# Autodesk Inventor assembly: Assembly ebeam heater IS v0
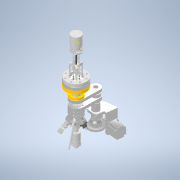
[picture p0: Inventor's stored thumbnail of the model, 180x180]
Saved by Autodesk Inventor 2020 (Build 240168000, 168)
## iProperties
Created: 2019-05-26
Part Number: Assembly ebeam heater IS v0
Document SubType Name: Assembly
Designer: isadmin
Mass: 1360.95 g
Surface Area: 5412.04 cm^2
Volume: 1345.69 cm^3
Density: 1.01134 g/cm^3
Author: isadmin
## Documents named in this file (42)
- C:\Users\ColinP\Documents\Inventor\igor\Assembly ebeam heater CP v3.iam
- Assembly ebeam heater IS v0.iam
- C:\Users\ColinP\Documents\Inventor\igor\block.ipt
- C:\Users\ColinP\Documents\Inventor\igor\Shutter.ipt
- C:\Users\ColinP\Documents\Inventor\igor\ceramic washer.ipt
- C:\Users\ColinP\Documents\Inventor\igor\Shielding.ipt
- C:\Users\ColinP\Documents\Inventor\igor\Bullet_v5_SiliconeSample.ipt
- C:\Users\ColinP\Documents\Inventor\igor\Bullet_v5_SiliconeSample_TopPart.ipt
- C:\Users\ColinP\Documents\Inventor\igor\670000.ipt
- C:\Users\ColinP\Documents\Inventor\igor\MCF275-FlgMplxr-Cr1A5_(53-321020-A).ipt
- C:\Users\ColinP\Documents\Inventor\igor\665501.ipt
- C:\Users\ColinP\Documents\Inventor\igor\rotatable rod table.ipt
- C:\Users\ColinP\Documents\Inventor\igor\updated table+legs.iam
- C:\Users\ColinP\Documents\Inventor\igor\square eyelet.ipt
- C:\Users\ColinP\Documents\Inventor\igor\buffer.ipt
- C:\Users\ColinP\Documents\Inventor\igor\4.5to2.75converotr.ipt
- C:\Users\ColinP\Documents\Inventor\igor\rotaryconnector.ipt
- C:\Users\ColinP\Documents\Inventor\igor\140007.ipt
- C:\Users\ColinP\Documents\Inventor\Content Center Files\R2020\en-US\ISO 4029\ISO 4029 - M2 x 2 - ISO.ipt
- C:\Users\ColinP\Documents\Inventor\igor\9312007.iam
- C:\Users\ColinP\Documents\Inventor\igor\eft0181032.ipt
- C:\Users\ColinP\Documents\Inventor\igor\filwasher.ipt
- C:\Users\ColinP\Documents\Inventor\igor\fileholddub.ipt
- C:\Users\ColinP\Documents\Inventor\Content Center Files\R2020\en-US\ISO 4017(1)\ISO 4017 - M2.5 x 5 - ISO.ipt
- C:\Users\ColinP\Documents\Inventor\igor\water.ipt
- C:\Users\ColinP\Documents\Inventor\igor\stability copy2.ipt
- C:\Users\ColinP\Documents\Inventor\igor\stability copy.ipt
- C:\Users\ColinP\Documents\Inventor\igor\shroud 2.ipt
- C:\Users\ColinP\Documents\Inventor\igor\4.5 rod.ipt
- C:\Users\ColinP\Documents\Inventor\igor\5011T170_WORM-DRIVE CLAMP FOR FIRM HOSE AND TUBE.ipt
- C:\Users\ColinP\Documents\Inventor\igor\filament.ipt
- C:\Users\ColinP\Documents\Inventor\Content Center Files\R2020\en-US\ISO 4032(2)\ISO 4032 - M3.5 - ISO.ipt
- C:\Users\ColinP\Documents\Inventor\igor\110001.ipt
- C:\Users\ColinP\Documents\Inventor\igor\waterpipe assembly.ipt
- C:\Users\ColinP\Documents\Inventor\igor\waterpipe assembly 2.ipt
- C:\Users\ColinP\Documents\Inventor\igor\waterpipe3.ipt
- C:\Users\ColinP\Documents\Inventor\igor\flange 4_5 double_sided.ipt
- C:\Users\ColinP\Downloads\SS-2-VCR-CG-SwagelokCompany-07-31-2019(1).ipt
- C:\Users\ColinP\Downloads\SS-2-VCR-1-2-SwagelokCompany-08-01-2019.ipt
- C:\Users\ColinP\Documents\Inventor\Content Center Files\R2020\en-US\ISO 4032(2)\ISO 4032 - M3 - ISO.ipt
- C:\Users\ColinP\Downloads\110021.ipt
- C:\Users\ColinP\Documents\Inventor\igor\part12.ipt
## Components (150 placed, 40 different names)
1. rotatable rod table:1 — Mate:48, Insert:171, Insert:173, Insert:174, Insert:175, Rigid:18, Insert:176, Insert:177, Insert:181, Insert:187, Mate:246, Insert:207, Mate:273, Mate:274
2. block for bullet:1 — Mate:249
3. Shutter:1
4. ceramic washer:1
5. ceramic washer:2
6. ceramic washer:3
7. ceramic washer:4
8. Shielding:1
9. ceramic washer:5
10. ceramic washer:6
11. ceramic washer:7
12. ceramic washer:8
13. Bullet_v5_SiliconeSample:1
14. Bullet_v5_SiliconeSample_TopPart:1
15. rotation_670000:1 — Rotational:3, Rigid:18
16. MCF275-FlgMplxr-Cr1A5_(53-321020-A):1 — Rotational:3, Rigid:5, Rotational:14, Rotational:16, Rigid:23, Rigid:24
17. zstage_665501:1 — Rigid:8, Cylindrical:1, Mate:235
18. 140007:1 — Rigid:5, Rigid:8, Insert:131, Insert:132, Insert:133, Insert:134, Insert:135, Insert:136, Mate:272, Mate:396, Mate:398
19. updated table+legs:1 [sub-assembly] — Mate:48, Mate:72, Rigid:14, Insert:166, Angle:1, Mate:215, Mate:216, Mate:217, Mate:218, Mate:219, Mate:220, Rotational:12, Rigid:22, Mate:241, Mate:250, Mate:254, Mate:278, Mate:281, Mate:288, Mate:290, Mate:292, Mate:294, Mate:296, Mate:298, Mate:300, Mate:302, Mate:304, Mate:306, Mate:308, Mate:310, Mate:312, Mate:314, Mate:316, Mate:318, Mate:320, Mate:322, Mate:324, Mate:326, Mate:328, Mate:330, Mate:332, Mate:334, Mate:336, Mate:338, Mate:340, Mate:342, Mate:344, Mate:346, Mate:348, Mate:350, Mate:352, Mate:354, Mate:356, Mate:358, Mate:360, Mate:362, Mate:364, Mate:366, Mate:368, Mate:370, Mate:404, Mate:406, Mate:408, Mate:430, Mate:432, Mate:434, Mate:436
20. buffer:4 — Insert:173
21. square eyelet:24 — Mate:327, Mate:339
22. square eyelet:25 — Mate:218, Mate:329, Mate:331
23. square eyelet:26 — Mate:325, Mate:337
24. buffer:5 — Insert:171
25. square eyelet:27 — Mate:349, Mate:363
26. square eyelet:28 — Mate:216, Mate:351, Mate:355
27. square eyelet:29 — Mate:353, Mate:357
28. buffer:6 — Insert:161, Insert:162, Insert:163, Insert:174
29. buffer:7 — Insert:176
30. square eyelet:33 — Mate:293, Mate:295
31. square eyelet:34 — Mate:220, Mate:297, Mate:299
32. square eyelet:35 — Mate:289, Mate:291
33. buffer:9 — Insert:177
34. square eyelet:39 — Mate:341, Mate:347
35. square eyelet:40 — Mate:217, Mate:333, Mate:343
36. square eyelet:41 — Mate:335, Mate:345
37. rotaryconnector:2 — Insert:149, Insert:150, Insert:151, Insert:152, Insert:187
38. square eyelet:49 — Insert:134, Mate:437
39. square eyelet:50 — Insert:135, Mate:435
40. square eyelet:51 — Insert:133, Insert:222
41. square eyelet:52 — Insert:131, Mate:72, Mate:433
42. square eyelet:53 — Insert:132, Mate:431
43. square eyelet:54 — Insert:136, Insert:223
44. buffer:10 — Insert:175
45. square eyelet:55 — Mate:215, Mate:315, Mate:323
46. square eyelet:56 — Mate:313, Mate:321
47. square eyelet:57 — Mate:317, Mate:319
48. 9312007:1 [sub-assembly] — Rotational:16
49. eft0181032:1 — Rigid:23
50. square eyelet:64 — Insert:162, Mate:301, Mate:303
51. square eyelet:65 — Insert:163, Mate:305, Mate:307
52. square eyelet:66 — Insert:161, Mate:219, Mate:309, Mate:311
53. filwasher:2 — Rigid:14, Insert:168, Rotational:12, Mate:279
54. fileholddub:1 — Insert:166, Rigid:17, Rotational:9, Angle:1
55. filwasher:5 — Rotational:9, Insert:169, Mate:280
56. filwasher:6 — Rigid:17, Insert:170, Mate:277
57. filwasher:7 — Insert:167, Rigid:22, Mate:276
58. buffer:11 — Insert:178, Insert:179, Insert:180, Insert:181
59. square eyelet:67 — Insert:178, Mate:361, Mate:367
60. square eyelet:68 — Insert:179, Mate:359, Mate:371
61. square eyelet:69 — Insert:180, Mate:254, Mate:365, Mate:369
62. ISO 4029 M2 x 2:1 — Insert:152
63. ISO 4029 M2 x 2:2 — Insert:150
64. ISO 4029 M2 x 2:3 — Insert:151
65. ISO 4029 M2 x 2:4 — Insert:149
66. ISO 4017 M2.5 x 5:1 — Insert:167
67. ISO 4017 M2.5 x 5:2 — Insert:168
68. ISO 4017 M2.5 x 5:3 — Insert:169
69. ISO 4017 M2.5 x 5:4 — Insert:170
70. water:1 — Insert:207, Insert:208, Insert:209, Insert:210, Flush:267, Mate:405, Mate:407, Mate:409, Mate:440, Mate:443, Insert:224, Insert:225
71. square eyelet:70 — Insert:210
72. square eyelet:71 — Insert:208, Mate:250
73. square eyelet:72 — Insert:209
74. 4.5to2.75converotr:1 — Cylindrical:1, Mate:235, Rigid:25
75. shroud 2:1 — Mate:241, Mate:249, Mate:264
76. 4.5 rod:1 — Mate:247, Mate:248, Insert:219
77. 4.5 rod:2 — Insert:221
78. 4.5 rod:3 — Insert:220
79. stability copy:1 — Insert:204, Insert:205, Insert:206, Mate:243, Mate:244, Mate:245, Mate:246
80. stability copy2:1 — Insert:205, Mate:244, Mate:247, Mate:248, Mate:286
81. stability copy2:2 — Insert:206, Mate:245, Mate:287
82. stability copy2:3 — Insert:204, Mate:243
83. 5011T170_WORM-DRIVE CLAMP FOR FIRM HOSE AND TUBE:1 — Mate:264, Flush:267
84. filament:1 — Mate:279, Mate:280, Mate:281
85. filament:2 — Mate:276, Mate:277, Mate:278
86. ISO 4032 M3.5:1 — Mate:288, Mate:289
87. ISO 4032 M3.5:2 — Mate:290, Mate:291
88. ISO 4032 M3.5:3 — Mate:292, Mate:293
89. ISO 4032 M3.5:4 — Mate:294, Mate:295
90. ISO 4032 M3.5:5 — Mate:296, Mate:297
91. ISO 4032 M3.5:6 — Mate:298, Mate:299
92. ISO 4032 M3.5:7 — Mate:300, Mate:301
93. ISO 4032 M3.5:8 — Mate:302, Mate:303
94. ISO 4032 M3.5:9 — Mate:304, Mate:305
95. ISO 4032 M3.5:10 — Mate:306, Mate:307
96. ISO 4032 M3.5:11 — Mate:308, Mate:309
97. ISO 4032 M3.5:12 — Mate:310, Mate:311
98. ISO 4032 M3.5:13 — Mate:312, Mate:313
99. ISO 4032 M3.5:14 — Mate:314, Mate:315
100. ISO 4032 M3.5:15 — Mate:316, Mate:317
101. ISO 4032 M3.5:16 — Mate:318, Mate:319
102. ISO 4032 M3.5:17 — Mate:320, Mate:321
103. ISO 4032 M3.5:18 — Mate:322, Mate:323
104. ISO 4032 M3.5:19 — Mate:324, Mate:325
105. ISO 4032 M3.5:20 — Mate:326, Mate:327
106. ISO 4032 M3.5:21 — Mate:328, Mate:329
107. ISO 4032 M3.5:22 — Mate:330, Mate:331
108. ISO 4032 M3.5:23 — Mate:332, Mate:333
109. ISO 4032 M3.5:24 — Mate:334, Mate:335
110. ISO 4032 M3.5:25 — Mate:336, Mate:337
111. ISO 4032 M3.5:26 — Mate:338, Mate:339
112. ISO 4032 M3.5:27 — Mate:340, Mate:341
113. ISO 4032 M3.5:28 — Mate:342, Mate:343
114. ISO 4032 M3.5:29 — Mate:344, Mate:345
115. ISO 4032 M3.5:30 — Mate:346, Mate:347
116. ISO 4032 M3.5:31 — Mate:348, Mate:349
117. ISO 4032 M3.5:32 — Mate:350, Mate:351
118. ISO 4032 M3.5:33 — Mate:352, Mate:353
119. ISO 4032 M3.5:34 — Mate:354, Mate:355
120. ISO 4032 M3.5:35 — Mate:356, Mate:357
121. ISO 4032 M3.5:36 — Mate:358, Mate:359
122. ISO 4032 M3.5:37 — Mate:360, Mate:361
123. ISO 4032 M3.5:38 — Mate:362, Mate:363
124. ISO 4032 M3.5:39 — Mate:364, Mate:365
125. ISO 4032 M3.5:40 — Mate:366, Mate:367
126. ISO 4032 M3.5:41 — Mate:368, Mate:369
127. ISO 4032 M3.5:42 — Mate:370, Mate:371
128. 110001:1 — Rotational:14, Mate:397
129. 110001:2 — Rigid:24, Mate:399
130. waterpipe assembly:1 — Mate:396, Mate:397, Mate:410, Mate:411, Mate:429
131. waterpipe assembly 2:1 — Mate:398, Mate:399, Mate:412, Mate:413, Mate:428
132. ISO 4032 M3.5:55 — Mate:404, Mate:405
133. ISO 4032 M3.5:56 — Mate:406, Mate:407
134. ISO 4032 M3.5:57 — Mate:408, Mate:409
135. waterpipe3:1 — Mate:410, Mate:411, Mate:429, Mate:439
136. waterpipe3:2 — Mate:412, Mate:413, Mate:428, Mate:438
137. flange 4_5 double_sided:1 — Rigid:25, Insert:219, Insert:220, Insert:221, Rigid:26
138. SS-2-VCR-CG-SwagelokCompany-07-31-2019(1):1 — Mate:418, Mate:419, Mate:439
139. SS-2-VCR-CG-SwagelokCompany-07-31-2019(1):2 — Mate:420, Mate:421, Mate:438
140. SS-2-VCR-1-2-SwagelokCompany-08-01-2019:1 — Mate:418, Mate:419, Mate:444
141. SS-2-VCR-1-2-SwagelokCompany-08-01-2019:2 — Mate:420, Mate:421, Mate:445
142. ISO 4032 M3.5:58 — Mate:430, Mate:431
143. ISO 4032 M3:1 — Insert:222
144. ISO 4032 M3.5:59 — Mate:432, Mate:433
145. ISO 4032 M3:2 — Insert:223
146. ISO 4032 M3:3 — Mate:434, Mate:435
147. ISO 4032 M3:4 — Mate:436, Mate:437
148. 110021:1 — Rigid:26
149. part12:1 — Mate:443, Insert:224, Mate:444, Symmetry:1
150. part12:2 — Mate:440, Insert:225, Mate:445, Symmetry:1
## Relationships (254: Mate 171, Insert 61, WeldJoint 10, RevoluteJoint 5, Flush 4, Angle 1, CylindricalJoint 1, Symmetry 1)
- [Mate]: block for bullet:1 ↔ Shutter:1
- [Mate]: block for bullet:1 ↔ Shutter:1
- [Mate]: block for bullet:1 ↔ Shutter:1
- [Mate]: block for bullet:1 ↔ ceramic washer:2
- [Mate]: block for bullet:1 ↔ ceramic washer:2
- [Mate]: block for bullet:1 ↔ ceramic washer:1
- [Mate]: block for bullet:1 ↔ ceramic washer:1
- [Mate]: block for bullet:1 ↔ ceramic washer:4
- [Mate]: block for bullet:1 ↔ ceramic washer:4
- [Mate]: block for bullet:1 ↔ ceramic washer:3
- [Mate]: block for bullet:1 ↔ ceramic washer:3
- [Mate]: ceramic washer:1 ↔ Shielding:1
- [Flush]: block for bullet:1 ↔ Shielding:1
- [Flush]: block for bullet:1 ↔ Shielding:1
- [Mate]: block for bullet:1 ↔ ceramic washer:5
- [Mate]: block for bullet:1 ↔ ceramic washer:5
- [Mate]: block for bullet:1 ↔ ceramic washer:6
- [Mate]: block for bullet:1 ↔ ceramic washer:6
- [Mate]: block for bullet:1 ↔ ceramic washer:7
- [Mate]: block for bullet:1 ↔ ceramic washer:7
- [Mate]: block for bullet:1 ↔ ceramic washer:8
- [Mate]: block for bullet:1 ↔ ceramic washer:8
- [Mate] (0.0254 mm): Bullet_v5_SiliconeSample:1 ↔ Bullet_v5_SiliconeSample_TopPart:1
- [Mate]: Bullet_v5_SiliconeSample:1 ↔ Bullet_v5_SiliconeSample_TopPart:1
- [Insert]: block for bullet:1 ↔ Bullet_v5_SiliconeSample:1
- [Insert]: rotatable rod table:1 ↔ block for bullet:1
- [Insert]: rotatable rod table:1 ↔ block for bullet:1
- [Insert]: buffer:4 ↔ square eyelet:25
- [Insert]: buffer:4 ↔ square eyelet:24
- [Insert]: buffer:4 ↔ square eyelet:26
- [Insert]: buffer:5 ↔ square eyelet:28
- [Insert]: buffer:5 ↔ square eyelet:27
- [Insert]: buffer:5 ↔ square eyelet:29
- [Insert]: buffer:7 ↔ square eyelet:34
- [Insert]: buffer:7 ↔ square eyelet:33
- [Insert]: buffer:7 ↔ square eyelet:35
- [Insert]: buffer:9 ↔ square eyelet:40
- [Insert]: buffer:9 ↔ square eyelet:39
- [Insert]: buffer:9 ↔ square eyelet:41
- Mate:48: rotatable rod table:1 ↔ updated table+legs:1
- Rotational:3 [RevoluteJoint]: rotation_670000:1 ↔ MCF275-FlgMplxr-Cr1A5_(53-321020-A):1
- Rigid:5 [WeldJoint]: MCF275-FlgMplxr-Cr1A5_(53-321020-A):1 ↔ 140007:1
- Rigid:8 [WeldJoint]: zstage_665501:1 ↔ 140007:1
- Insert:131: 140007:1 ↔ square eyelet:52
- Insert:132: 140007:1 ↔ square eyelet:53
- Insert:133: 140007:1 ↔ square eyelet:51
- Insert:134: 140007:1 ↔ square eyelet:49
- Insert:135: 140007:1 ↔ square eyelet:50
- Insert:136: 140007:1 ↔ square eyelet:54
- [Insert]: buffer:10 ↔ square eyelet:56
- [Insert]: buffer:10 ↔ square eyelet:55
- [Insert]: buffer:10 ↔ square eyelet:57
- Insert:149: rotaryconnector:2 ↔ ISO 4029 M2 x 2:4
- Insert:150: rotaryconnector:2 ↔ ISO 4029 M2 x 2:2
- Insert:151: rotaryconnector:2 ↔ ISO 4029 M2 x 2:3
- Insert:152: rotaryconnector:2 ↔ ISO 4029 M2 x 2:1
- Mate:72: updated table+legs:1 ↔ square eyelet:52
- Insert:161: buffer:6 ↔ square eyelet:66
- Insert:162: buffer:6 ↔ square eyelet:64
- Insert:163: buffer:6 ↔ square eyelet:65
- Rigid:14 [WeldJoint]: updated table+legs:1 ↔ filwasher:2
- Insert:166 (-6.35 mm): updated table+legs:1 ↔ fileholddub:1
- Rigid:17 [WeldJoint]: fileholddub:1 ↔ filwasher:6
- Rotational:9 [RevoluteJoint]: fileholddub:1 ↔ filwasher:5
- Insert:167: filwasher:7 ↔ ISO 4017 M2.5 x 5:1
- Insert:168: filwasher:2 ↔ ISO 4017 M2.5 x 5:2
- Insert:169: filwasher:5 ↔ ISO 4017 M2.5 x 5:3
- Insert:170: filwasher:6 ↔ ISO 4017 M2.5 x 5:4
- Insert:171 (175.895 mm): rotatable rod table:1 ↔ buffer:5
- Insert:173 (199.644 mm): rotatable rod table:1 ↔ buffer:4
- Insert:174 (223.52 mm): rotatable rod table:1 ↔ buffer:6
- Insert:175 (211.455 mm): rotatable rod table:1 ↔ buffer:10
- Angle:1 (180 deg): updated table+legs:1 ↔ fileholddub:1
- Rigid:18 [WeldJoint]: rotatable rod table:1 ↔ rotation_670000:1
- Insert:176 (235.585 mm): rotatable rod table:1 ↔ buffer:7
- Insert:177 (187.96 mm): rotatable rod table:1 ↔ buffer:9
- Insert:178: buffer:11 ↔ square eyelet:67
- Insert:179: buffer:11 ↔ square eyelet:68
- Insert:180: buffer:11 ↔ square eyelet:69
- Insert:181 (163.83 mm): rotatable rod table:1 ↔ buffer:11
- Insert:187 (-12.7 mm): rotatable rod table:1 ↔ rotaryconnector:2
- Cylindrical:1: zstage_665501:1 ↔ 4.5to2.75converotr:1
- Mate:215: updated table+legs:1 ↔ square eyelet:55
- Mate:216: updated table+legs:1 ↔ square eyelet:28
- Mate:217: updated table+legs:1 ↔ square eyelet:40
- Mate:218: updated table+legs:1 ↔ square eyelet:25
- Mate:219: updated table+legs:1 ↔ square eyelet:66
- Mate:220: updated table+legs:1 ↔ square eyelet:34
- Rotational:12 [RevoluteJoint]: updated table+legs:1 ↔ filwasher:2
- Rigid:22 [WeldJoint]: updated table+legs:1 ↔ filwasher:7
- Mate:235: zstage_665501:1 ↔ 4.5to2.75converotr:1
- Mate:241: updated table+legs:1 ↔ shroud 2:1
- Insert:204: stability copy:1 ↔ stability copy2:3
- Insert:205: stability copy:1 ↔ stability copy2:1
- Insert:206: stability copy:1 ↔ stability copy2:2
- Mate:243: stability copy:1 ↔ stability copy2:3
- Mate:244: stability copy:1 ↔ stability copy2:1
- Mate:245: stability copy:1 ↔ stability copy2:2
- Mate:246: rotatable rod table:1 ↔ stability copy:1
- Mate:247: 4.5 rod:1 ↔ stability copy2:1
- Mate:248: 4.5 rod:1 ↔ stability copy2:1
- Mate:249: block for bullet:1 ↔ shroud 2:1
- Insert:207 (27.94 mm): rotatable rod table:1 ↔ water:1
- Insert:208: water:1 ↔ square eyelet:71
- Insert:209: water:1 ↔ square eyelet:72
- Insert:210: water:1 ↔ square eyelet:70
- Mate:250: updated table+legs:1 ↔ square eyelet:71
- Mate:254: updated table+legs:1 ↔ square eyelet:69
- Mate:264: shroud 2:1 ↔ 5011T170_WORM-DRIVE CLAMP FOR FIRM HOSE AND TUBE:1
- Mate:272: 140007:1
- Mate:273: rotatable rod table:1
- Mate:274: rotatable rod table:1
- Mate:276: filwasher:7 ↔ filament:2
- Mate:277: filwasher:6 ↔ filament:2
- Mate:278: updated table+legs:1 ↔ filament:2
- Mate:279: filwasher:2 ↔ filament:1
- Mate:280: filwasher:5 ↔ filament:1
- Mate:281: updated table+legs:1 ↔ filament:1
- Mate:286: stability copy2:1
- Mate:287: stability copy2:2
- Mate:288: updated table+legs:1 ↔ ISO 4032 M3.5:1
- Mate:289: square eyelet:35 ↔ ISO 4032 M3.5:1
- Mate:290: updated table+legs:1 ↔ ISO 4032 M3.5:2
- Mate:291: square eyelet:35 ↔ ISO 4032 M3.5:2
- Mate:292: updated table+legs:1 ↔ ISO 4032 M3.5:3
- Mate:293: square eyelet:33 ↔ ISO 4032 M3.5:3
- Mate:294: updated table+legs:1 ↔ ISO 4032 M3.5:4
- Mate:295: square eyelet:33 ↔ ISO 4032 M3.5:4
- Mate:296: updated table+legs:1 ↔ ISO 4032 M3.5:5
- Mate:297: square eyelet:34 ↔ ISO 4032 M3.5:5
- Mate:298: updated table+legs:1 ↔ ISO 4032 M3.5:6
- Mate:299: square eyelet:34 ↔ ISO 4032 M3.5:6
- Mate:300: updated table+legs:1 ↔ ISO 4032 M3.5:7
- Mate:301: square eyelet:64 ↔ ISO 4032 M3.5:7
- Mate:302: updated table+legs:1 ↔ ISO 4032 M3.5:8
- Mate:303: square eyelet:64 ↔ ISO 4032 M3.5:8
- Mate:304: updated table+legs:1 ↔ ISO 4032 M3.5:9
- Mate:305: square eyelet:65 ↔ ISO 4032 M3.5:9
- Mate:306: updated table+legs:1 ↔ ISO 4032 M3.5:10
- Mate:307: square eyelet:65 ↔ ISO 4032 M3.5:10
- Mate:308: updated table+legs:1 ↔ ISO 4032 M3.5:11
- Mate:309: square eyelet:66 ↔ ISO 4032 M3.5:11
- Mate:310: updated table+legs:1 ↔ ISO 4032 M3.5:12
- Mate:311: square eyelet:66 ↔ ISO 4032 M3.5:12
- Mate:312: updated table+legs:1 ↔ ISO 4032 M3.5:13
- Mate:313: square eyelet:56 ↔ ISO 4032 M3.5:13
- Mate:314: updated table+legs:1 ↔ ISO 4032 M3.5:14
- Mate:315: square eyelet:55 ↔ ISO 4032 M3.5:14
- Mate:316: updated table+legs:1 ↔ ISO 4032 M3.5:15
- Mate:317: square eyelet:57 ↔ ISO 4032 M3.5:15
- Mate:318: updated table+legs:1 ↔ ISO 4032 M3.5:16
- Mate:319: square eyelet:57 ↔ ISO 4032 M3.5:16
- Mate:320: updated table+legs:1 ↔ ISO 4032 M3.5:17
- Mate:321: square eyelet:56 ↔ ISO 4032 M3.5:17
- Mate:322: updated table+legs:1 ↔ ISO 4032 M3.5:18
- Mate:323: square eyelet:55 ↔ ISO 4032 M3.5:18
- Mate:324: updated table+legs:1 ↔ ISO 4032 M3.5:19
- Mate:325: square eyelet:26 ↔ ISO 4032 M3.5:19
- Mate:326: updated table+legs:1 ↔ ISO 4032 M3.5:20
- Mate:327: square eyelet:24 ↔ ISO 4032 M3.5:20
- Mate:328: updated table+legs:1 ↔ ISO 4032 M3.5:21
- Mate:329: square eyelet:25 ↔ ISO 4032 M3.5:21
- Mate:330: updated table+legs:1 ↔ ISO 4032 M3.5:22
- Mate:331: square eyelet:25 ↔ ISO 4032 M3.5:22
- Mate:332: updated table+legs:1 ↔ ISO 4032 M3.5:23
- Mate:333: square eyelet:40 ↔ ISO 4032 M3.5:23
- Mate:334: updated table+legs:1 ↔ ISO 4032 M3.5:24
- Mate:335: square eyelet:41 ↔ ISO 4032 M3.5:24
- Mate:336: updated table+legs:1 ↔ ISO 4032 M3.5:25
- Mate:337: square eyelet:26 ↔ ISO 4032 M3.5:25
- Mate:338: updated table+legs:1 ↔ ISO 4032 M3.5:26
- Mate:339: square eyelet:24 ↔ ISO 4032 M3.5:26
- Mate:340: updated table+legs:1 ↔ ISO 4032 M3.5:27
- Mate:341: square eyelet:39 ↔ ISO 4032 M3.5:27
- Mate:342: updated table+legs:1 ↔ ISO 4032 M3.5:28
- Mate:343: square eyelet:40 ↔ ISO 4032 M3.5:28
- Mate:344: updated table+legs:1 ↔ ISO 4032 M3.5:29
- Mate:345: square eyelet:41 ↔ ISO 4032 M3.5:29
- Mate:346: updated table+legs:1 ↔ ISO 4032 M3.5:30
- Mate:347: square eyelet:39 ↔ ISO 4032 M3.5:30
- Mate:348: updated table+legs:1 ↔ ISO 4032 M3.5:31
- Mate:349: square eyelet:27 ↔ ISO 4032 M3.5:31
- Mate:350: updated table+legs:1 ↔ ISO 4032 M3.5:32
- Mate:351: square eyelet:28 ↔ ISO 4032 M3.5:32
- Mate:352: updated table+legs:1 ↔ ISO 4032 M3.5:33
- Mate:353: square eyelet:29 ↔ ISO 4032 M3.5:33
- Mate:354: updated table+legs:1 ↔ ISO 4032 M3.5:34
- Mate:355: square eyelet:28 ↔ ISO 4032 M3.5:34
- Mate:356: updated table+legs:1 ↔ ISO 4032 M3.5:35
- Mate:357: square eyelet:29 ↔ ISO 4032 M3.5:35
- Mate:358: updated table+legs:1 ↔ ISO 4032 M3.5:36
- Mate:359: square eyelet:68 ↔ ISO 4032 M3.5:36
- Mate:360: updated table+legs:1 ↔ ISO 4032 M3.5:37
- Mate:361: square eyelet:67 ↔ ISO 4032 M3.5:37
- Mate:362: updated table+legs:1 ↔ ISO 4032 M3.5:38
- Mate:363: square eyelet:27 ↔ ISO 4032 M3.5:38
- Mate:364: updated table+legs:1 ↔ ISO 4032 M3.5:39
- Mate:365: square eyelet:69 ↔ ISO 4032 M3.5:39
- Mate:366: updated table+legs:1 ↔ ISO 4032 M3.5:40
- Mate:367: square eyelet:67 ↔ ISO 4032 M3.5:40
- Mate:368: updated table+legs:1 ↔ ISO 4032 M3.5:41
- Mate:369: square eyelet:69 ↔ ISO 4032 M3.5:41
- Mate:370: updated table+legs:1 ↔ ISO 4032 M3.5:42
- Mate:371: square eyelet:68 ↔ ISO 4032 M3.5:42
- Rotational:14 [RevoluteJoint]: MCF275-FlgMplxr-Cr1A5_(53-321020-A):1 ↔ 110001:1
- Rotational:16 [RevoluteJoint]: MCF275-FlgMplxr-Cr1A5_(53-321020-A):1 ↔ 9312007:1
- Rigid:23 [WeldJoint]: MCF275-FlgMplxr-Cr1A5_(53-321020-A):1 ↔ eft0181032:1
- Rigid:24 [WeldJoint]: MCF275-FlgMplxr-Cr1A5_(53-321020-A):1 ↔ 110001:2
- Flush:3 (3.175 mm)
- Mate:396: 140007:1 ↔ waterpipe assembly:1
- Mate:397: 110001:1 ↔ waterpipe assembly:1
- Mate:398: 140007:1 ↔ waterpipe assembly 2:1
- Mate:399: 110001:2 ↔ waterpipe assembly 2:1
- Flush:267: water:1 ↔ 5011T170_WORM-DRIVE CLAMP FOR FIRM HOSE AND TUBE:1
- Mate:404: updated table+legs:1 ↔ ISO 4032 M3.5:55
- Mate:405: water:1 ↔ ISO 4032 M3.5:55
- Mate:406: updated table+legs:1 ↔ ISO 4032 M3.5:56
- Mate:407: water:1 ↔ ISO 4032 M3.5:56
- Mate:408: updated table+legs:1 ↔ ISO 4032 M3.5:57
- Mate:409: water:1 ↔ ISO 4032 M3.5:57
- Mate:410: waterpipe assembly:1 ↔ waterpipe3:1
- Mate:411: waterpipe assembly:1 ↔ waterpipe3:1
- Mate:412: waterpipe assembly 2:1 ↔ waterpipe3:2
- Mate:413: waterpipe assembly 2:1 ↔ waterpipe3:2
- Rigid:25 [WeldJoint]: 4.5to2.75converotr:1 ↔ flange 4_5 double_sided:1
- Insert:219: 4.5 rod:1 ↔ flange 4_5 double_sided:1
- Insert:220: 4.5 rod:3 ↔ flange 4_5 double_sided:1
- Insert:221: 4.5 rod:2 ↔ flange 4_5 double_sided:1
- Mate:418: SS-2-VCR-CG-SwagelokCompany-07-31-2019(1):1 ↔ SS-2-VCR-1-2-SwagelokCompany-08-01-2019:1
- Mate:419: SS-2-VCR-CG-SwagelokCompany-07-31-2019(1):1 ↔ SS-2-VCR-1-2-SwagelokCompany-08-01-2019:1
- Mate:420: SS-2-VCR-CG-SwagelokCompany-07-31-2019(1):2 ↔ SS-2-VCR-1-2-SwagelokCompany-08-01-2019:2
- Mate:421: SS-2-VCR-CG-SwagelokCompany-07-31-2019(1):2 ↔ SS-2-VCR-1-2-SwagelokCompany-08-01-2019:2
- Mate:428: waterpipe assembly 2:1 ↔ waterpipe3:2
- Mate:429: waterpipe assembly:1 ↔ waterpipe3:1
- Mate:430: updated table+legs:1 ↔ ISO 4032 M3.5:58
- Mate:431: square eyelet:53 ↔ ISO 4032 M3.5:58
- Insert:222: square eyelet:51 ↔ ISO 4032 M3:1
- Mate:432: updated table+legs:1 ↔ ISO 4032 M3.5:59
- Mate:433: square eyelet:52 ↔ ISO 4032 M3.5:59
- Insert:223: square eyelet:54 ↔ ISO 4032 M3:2
- Mate:434: updated table+legs:1 ↔ ISO 4032 M3:3
- Mate:435: square eyelet:50 ↔ ISO 4032 M3:3
- Mate:436: updated table+legs:1 ↔ ISO 4032 M3:4
- Mate:437: square eyelet:49 ↔ ISO 4032 M3:4
- Mate:438: waterpipe3:2 ↔ SS-2-VCR-CG-SwagelokCompany-07-31-2019(1):2
- Mate:439: waterpipe3:1 ↔ SS-2-VCR-CG-SwagelokCompany-07-31-2019(1):1
- Mate:440: water:1 ↔ part12:2
- Mate:443: water:1 ↔ part12:1
- Insert:224 (-11.43 mm): water:1 ↔ part12:1
- Insert:225 (-11.43 mm): water:1 ↔ part12:2
- Mate:444: SS-2-VCR-1-2-SwagelokCompany-08-01-2019:1 ↔ part12:1
- Mate:445: SS-2-VCR-1-2-SwagelokCompany-08-01-2019:2 ↔ part12:2
- Symmetry:1: part12:1 ↔ part12:2
- Rigid:26 [WeldJoint]: flange 4_5 double_sided:1 ↔ 110021:1
## Named parameters: d75_d58 = 0 mm, d76_d19 = 0 mm, d77_d22_d25 = 0 mm, d78_d23_d26 = 0 mm, d79_d24_d35 = 0 mm, d80_d25_d36 = 0 mm, d81_d26_d37 = 0 mm, d82_d27_d38 = 0 mm, d83_d28_d39 = 0 mm, d84_d29_d40 = 0 mm, d85_d30_d41 = 0 mm, d86_d31_d42 = 0 mm, d87_d43 = 0 mm, d88_d44 = 0 mm, d89_d45 = 0 mm, d90_d46 = 0 mm, d91_d47 = 0 mm, d92_d48 = 0 mm, d93_d49 = 0 mm, d94_d50 = 0 mm, d95_d51 = 0 mm, d96_d52 = 0 mm, d97_d53 = 0 mm, d98_d56_d0 = 0.0254 mm, d99_d57_d1 = 0 mm, d148_d124_d114_d111 = 0 mm, d149_d125_d115_d112 = 0 mm, d150_d126_d116_d113 = 0 mm, d152_d124_d114_d111 = 0 mm, d153_d125_d115_d112 = 0 mm, d154_d126_d116_d113 = 0 mm, d163_d124_d114_d111 = 0 mm, d164_d125_d115_d112 = 0 mm, d165_d126_d116_d113 = 0 mm, d175_d111 = 0 mm, d176_d112 = 0 mm, d177_d113 = 0 mm, d314_d124_d114_d111 = 0 mm, d315_d125_d115_d112 = 0 mm, d316_d126_d116_d113 = 0 mm, sa_0 = 444.822
note: some values were not read from the file. Shown as the stored number, unit unknown: "sa_0".
